# Autodesk Inventor assembly: unit
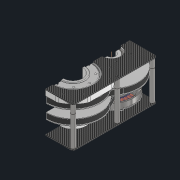
[picture p0: Inventor's stored thumbnail of the model, 180x180]
Saved by Autodesk Inventor 2022 (Build 260153000, 153)
## iProperties
Created: 2021-09-16
Part Number: unit
Document SubType Name: Assembly
Designer: Yuta Kage
Author: Yuta Kage
## Documents named in this file (23)
- C:\Users\yuta0\Documents\GitHub\catchrobo_hardware\model_v2\unit.iam
- C:\Users\yuta0\Documents\GitHub\catchrobo_hardware\model_v2\base1.ipt
- C:\Users\yuta0\Documents\GitHub\catchrobo_hardware\model_v2\base2.ipt
- C:\Users\yuta0\Documents\GitHub\catchrobo_hardware\assy-robot\ex8108.iam
- C:\Users\yuta0\Documents\GitHub\zebra_hardware\hardware\zebra_cad_v1.0\B6806ZZ.ipt
- C:\Users\yuta0\Documents\GitHub\catchrobo_hardware\assy-robot\B6815ZZ.ipt
- C:\Users\yuta0\Documents\GitHub\catchrobo_hardware\model_v2\base4.ipt
- C:\Users\yuta0\Documents\GitHub\catchrobo_hardware\assy-robot\s-assy-driver.iam
- C:\Users\yuta0\Documents\GitHub\catchrobo_hardware\model_v2\carbonplate1.ipt
- C:\Users\yuta0\Documents\GitHub\catchrobo_hardware\model_v2\base5.ipt
- C:\Users\yuta0\Documents\GitHub\catchrobo_hardware\assy-robot\ARF-4_1.ipt
- C:\Users\yuta0\Documents\GitHub\catchrobo_hardware\model_v2\base6.ipt
- C:\Users\yuta0\Documents\GitHub\catchrobo_hardware\model_v2\CSHELH-SUS-M3-25.ipt
- C:\Users\yuta0\Downloads\P&G\P&G\CB3-25.ipt
- C:\Users\yuta0\Documents\GitHub\catchrobo_hardware\assy-robot\LBNR3.ipt
- C:\Users\yuta0\Documents\GitHub\catchrobo_hardware\model_v2\base7.ipt
- C:\Users\yuta0\Documents\GitHub\catchrobo_hardware\assy-robot\s-assy-unit-magnet_2.iam
- C:\Users\yuta0\Documents\GitHub\catchrobo_hardware\assy-robot\B688ZZ.ipt
- C:\Users\yuta0\Documents\GitHub\catchrobo_hardware\model_v2\belt_2.ipt
- C:\Users\yuta0\Documents\GitHub\catchrobo_hardware\model_v2\carbonplate3.ipt
- C:\Users\yuta0\Documents\GitHub\catchrobo_hardware\assy-robot\ARF-4_2.ipt
- C:\Users\yuta0\Documents\GitHub\catchrobo_hardware\model_v2\CF-417E.ipt
- C:\Users\yuta0\Documents\GitHub\catchrobo_hardware\assy-robot\CB4-6.ipt
## Components (56 placed, 22 different names)
1. base2:1 — メイト:1, メイト:2, メイト:3, メイト:4, メイト:5, メイト:51, メイト:52
2. base7:1 — メイト:10, メイト:11, メイト:38, メイト:39, メイト:73, メイト:82, メイト:83
3. B6806ZZ:1 — メイト:4, メイト:5, メイト:10, メイト:11
4. ex8108:3 [sub-assembly] — メイト:1, メイト:2, メイト:3, メイト:35, メイト:36, メイト:37, メイト:59, メイト:60, メイト:61, メイト:63, メイト:84
5. B6815ZZ:1 — メイト:16, メイト:17, メイト:40
6. base1:1 — メイト:16, メイト:17, メイト:22, メイト:23, メイト:70
7. B6806ZZ:2 — メイト:18, メイト:19, メイト:50
8. base4:1 — メイト:18, メイト:19, メイト:20, メイト:21, メイト:53, メイト:74, メイト:76
9. B6806ZZ:3 — メイト:20, メイト:21, メイト:22, メイト:23
10. carbonplate1:3 — メイト:35, メイト:36, メイト:37, メイト:44, メイト:56, メイト:64, メイト:68, メイト:77, メイト:79, メイト:80, メイト:81, メイト:89, メイト:90, メイト:98, メイト:102, メイト:103, メイト:106, メイト:107, メイト:109, メイト:110
11. B6806ZZ:4 — メイト:38, メイト:39, メイト:41, メイト:42
12. base5:1 — メイト:40, メイト:41, メイト:42, メイト:45, メイト:91
13. ARF-4_1:1 — メイト:44, メイト:77, メイト:95
14. base6:1 — メイト:50, メイト:53, メイト:55, メイト:58, メイト:68, メイト:69, メイト:75
15. s-assy-unit-magnet_2:1 [sub-assembly] — メイト:59, メイト:60, メイト:61, メイト:62
16. s-assy-driver:2 [sub-assembly] — メイト:62, メイト:63, メイト:64
17. belt_2:1 — メイト:75, メイト:76, メイト:84, メイト:88, フラッシュ:1
18. belt_2:2 — メイト:69, メイト:70, メイト:83, フラッシュ:3
19. belt_2:3 — メイト:73, メイト:74, メイト:82, フラッシュ:2
20. ARF-4_2:1 — メイト:79, メイト:85, メイト:86, メイト:87
21. ARF-4_1:3 — メイト:80, メイト:81, メイト:97
22. carbonplate3:1 — メイト:89, メイト:90, メイト:91, メイト:92, メイト:94, メイト:96, メイト:100
23. ARF-4_1:4 — メイト:92, メイト:98, メイト:99
24. CF-417E:1 — メイト:94, メイト:95
25. CF-417E:2 — メイト:96, メイト:97
26. CF-417E:3 — メイト:99, メイト:100
27. ARF-4_1:5 — メイト:102, メイト:103, メイト:104
28. CF-417E:4 — メイト:104
29. ARF-4_1:6 — メイト:106, メイト:107, メイト:108
30. CF-417E:5 — メイト:108
31. CSHELH-SUS-M3-25:2 — メイト:51, メイト:52
32. CSHELH-SUS-M3-25:3
33. CSHELH-SUS-M3-25:4
34. CSHELH-SUS-M3-25:5
35. CB3-25:1 — メイト:55, メイト:56, メイト:57
36. LBNR3:1 — メイト:57, メイト:58
37. CB3-25:2
38. LBNR3:2
39. CB3-25:3
40. LBNR3:3
41. CB3-25:4
42. LBNR3:4
43. CB3-25:5
44. LBNR3:5
45. CB3-25:6
46. LBNR3:6
47. B688ZZ:1 — メイト:85, メイト:88, フラッシュ:1
48. B688ZZ:2 — メイト:86, フラッシュ:2
49. B688ZZ:3 — メイト:87, フラッシュ:3
50. B688ZZ:4
51. B688ZZ:5
52. B688ZZ:6
53. CB4-6:1 — メイト:109, メイト:110
54. CB4-6:2
55. CB4-6:3
56. CB4-6:4
## Component patterns: (4 elements, first: CSHELH-SUS-M3-25:2), (6 elements, first: CB3-25:1 + LBNR3:1), (2 elements, first: B688ZZ:1 + B688ZZ:2 + B688ZZ:3), (4 elements, first: CB4-6:1)
## Relationships (81: Mate 78, Flush 3)
- メイト:1 [Mate]: base2:1 ↔ ex8108:3
- メイト:2 [Mate]: base2:1 ↔ ex8108:3
- メイト:3 [Mate]: base2:1 ↔ ex8108:3
- メイト:4 [Mate]: base2:1 ↔ B6806ZZ:1
- メイト:5 [Mate]: base2:1 ↔ B6806ZZ:1
- メイト:10 [Mate]: base7:1 ↔ B6806ZZ:1
- メイト:11 [Mate]: base7:1 ↔ B6806ZZ:1
- メイト:16 [Mate]: B6815ZZ:1 ↔ base1:1
- メイト:17 [Mate]: B6815ZZ:1 ↔ base1:1
- メイト:18 [Mate]: B6806ZZ:2 ↔ base4:1
- メイト:19 [Mate]: B6806ZZ:2 ↔ base4:1
- メイト:20 [Mate]: base4:1 ↔ B6806ZZ:3
- メイト:21 [Mate]: base4:1 ↔ B6806ZZ:3
- メイト:22 [Mate]: base1:1 ↔ B6806ZZ:3
- メイト:23 [Mate]: base1:1 ↔ B6806ZZ:3
- メイト:35 [Mate]: ex8108:3 ↔ carbonplate1:3
- メイト:36 [Mate]: ex8108:3 ↔ carbonplate1:3
- メイト:37 [Mate]: ex8108:3 ↔ carbonplate1:3
- メイト:38 [Mate]: base7:1 ↔ B6806ZZ:4
- メイト:39 [Mate]: base7:1 ↔ B6806ZZ:4
- メイト:40 [Mate]: B6815ZZ:1 ↔ base5:1
- メイト:41 [Mate]: B6806ZZ:4 ↔ base5:1
- メイト:42 [Mate]: B6806ZZ:4 ↔ base5:1
- メイト:44 [Mate]: carbonplate1:3 ↔ ARF-4_1:1
- メイト:45 [Mate]: base5:1
- メイト:50 [Mate]: B6806ZZ:2 ↔ base6:1
- メイト:51 [Mate]: base2:1 ↔ CSHELH-SUS-M3-25:2
- メイト:52 [Mate]: base2:1 ↔ CSHELH-SUS-M3-25:2
- メイト:53 [Mate]: base4:1 ↔ base6:1
- メイト:55 [Mate]: base6:1 ↔ CB3-25:1
- メイト:56 [Mate]: carbonplate1:3 ↔ CB3-25:1
- メイト:57 [Mate]: CB3-25:1 ↔ LBNR3:1
- メイト:58 [Mate]: base6:1 ↔ LBNR3:1
- メイト:59 [Mate]: ex8108:3 ↔ s-assy-unit-magnet_2:1
- メイト:60 [Mate]: ex8108:3 ↔ s-assy-unit-magnet_2:1
- メイト:61 [Mate]: ex8108:3 ↔ s-assy-unit-magnet_2:1
- メイト:62 [Mate]: s-assy-unit-magnet_2:1 ↔ s-assy-driver:2
- メイト:63 [Mate]: ex8108:3 ↔ s-assy-driver:2
- メイト:64 [Mate]: carbonplate1:3 ↔ s-assy-driver:2
- メイト:68 [Mate]: carbonplate1:3 ↔ base6:1
- メイト:69 [Mate]: base6:1 ↔ belt_2:2
- メイト:70 [Mate] (0.5 mm): base1:1 ↔ belt_2:2
- メイト:73 [Mate] (0.5 mm): base7:1 ↔ belt_2:3
- メイト:74 [Mate]: base4:1 ↔ belt_2:3
- メイト:75 [Mate]: base6:1 ↔ belt_2:1
- メイト:76 [Mate] (0.5 mm): base4:1 ↔ belt_2:1
- メイト:77 [Mate]: carbonplate1:3 ↔ ARF-4_1:1
- メイト:79 [Mate]: carbonplate1:3 ↔ ARF-4_2:1
- メイト:80 [Mate]: carbonplate1:3 ↔ ARF-4_1:3
- メイト:81 [Mate]: carbonplate1:3 ↔ ARF-4_1:3
- メイト:82 [Mate]: base7:1 ↔ belt_2:3
- メイト:83 [Mate]: base7:1 ↔ belt_2:2
- メイト:84 [Mate]: ex8108:3 ↔ belt_2:1
- メイト:85 [Mate]: ARF-4_2:1 ↔ B688ZZ:1
- メイト:86 [Mate]: ARF-4_2:1 ↔ B688ZZ:2
- メイト:87 [Mate]: ARF-4_2:1 ↔ B688ZZ:3
- メイト:88 [Mate]: belt_2:1 ↔ B688ZZ:1
- フラッシュ:1 [Flush]: belt_2:1 ↔ B688ZZ:1
- フラッシュ:2 [Flush]: belt_2:3 ↔ B688ZZ:2
- フラッシュ:3 [Flush]: belt_2:2 ↔ B688ZZ:3
- メイト:89 [Mate]: carbonplate1:3 ↔ carbonplate3:1
- メイト:90 [Mate]: carbonplate1:3 ↔ carbonplate3:1
- メイト:91 [Mate]: base5:1 ↔ carbonplate3:1
- メイト:92 [Mate]: carbonplate3:1 ↔ ARF-4_1:4
- メイト:94 [Mate]: carbonplate3:1 ↔ CF-417E:1
- メイト:95 [Mate]: ARF-4_1:1 ↔ CF-417E:1
- メイト:96 [Mate]: carbonplate3:1 ↔ CF-417E:2
- メイト:97 [Mate]: ARF-4_1:3 ↔ CF-417E:2
- メイト:98 [Mate]: carbonplate1:3 ↔ ARF-4_1:4
- メイト:99 [Mate]: ARF-4_1:4 ↔ CF-417E:3
- メイト:100 [Mate]: carbonplate3:1 ↔ CF-417E:3
- [Mate]: ARF-4_1:5 ↔ CF-417E:4
- メイト:102 [Mate]: carbonplate1:3 ↔ ARF-4_1:5
- メイト:103 [Mate]: carbonplate1:3 ↔ ARF-4_1:5
- メイト:104 [Mate]: ARF-4_1:5 ↔ CF-417E:4
- [Mate]: ARF-4_1:6 ↔ CF-417E:5
- メイト:106 [Mate]: carbonplate1:3 ↔ ARF-4_1:6
- メイト:107 [Mate]: carbonplate1:3 ↔ ARF-4_1:6
- メイト:108 [Mate]: ARF-4_1:6 ↔ CF-417E:5
- メイト:109 [Mate]: carbonplate1:3 ↔ CB4-6:1
- メイト:110 [Mate]: carbonplate1:3 ↔ CB4-6:1
## Named parameters: d124_d120 = 0 mm, d128_d120 = 0 mm
